# Autodesk Inventor assembly: proxxon_assembly
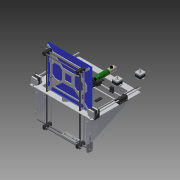
[picture p0: Inventor's stored thumbnail of the model, 180x180]
Saved by Autodesk Inventor 2013 (Build 170138000, 138)
## iProperties
Created: 2013-11-17
Part Number: proxxon_assembly
Document SubType Name: Assembly
Designer: Masta
Author: Masta
## Documents named in this file (24)
- D:\prusa i3\assembly\proxxon_assembly.iam
- D:\prusa i3\assembly\lasercut_aluminium\caddy.ipt
- D:\prusa i3\assembly\lasercut_aluminium\main_frame.ipt
- D:\prusa i3\assembly\lasercut_aluminium\side_frame.ipt
- D:\prusa i3\assembly\other\fi8x320.ipt
- D:\prusa i3\assembly\other\fi8x500.ipt
- D:\prusa i3\assembly\other\M5x300.ipt
- D:\prusa i3\assembly\other\M10x530.ipt
- D:\prusa i3\assembly\other\haetbed300.ipt
- D:\prusa i3\assembly\plastics\Y_corner.ipt
- D:\prusa i3\assembly\other\M8x290.ipt
- D:\prusa i3\assembly\other\M8x410.ipt
- D:\prusa i3\assembly\other\LM08UU.ipt
- D:\prusa i3\assembly\plastics\Prusa_i3_X_Carriage_Belt_Clamp.ipt
- D:\prusa i3\assembly\plastics\Prusa_i3_Y_Idler.ipt
- D:\prusa i3\assembly\other\nema17.ipt
- D:\prusa i3\assembly\old_parts_plastics\Prusa_i3_X_End_Idler.ipt
- D:\prusa i3\assembly\old_parts_plastics\Prusa_i3_X_End_Motor.ipt
- D:\prusa i3\assembly\old_parts_plastics\z-axis.ipt
- D:\prusa i3\assembly\old_parts_plastics\z-axis2.ipt
- D:\prusa i3\assembly\old_parts_plastics\x-carriage-24to30-gt2.ipt
- D:\prusa i3\assembly\plastics\adapter_50mm.ipt
- D:\prusa i3\assembly\old_parts_plastics\proxxon_mount.ipt
- D:\prusa i3\assembly\other\proxxon.ipt
## Components (48 placed, 23 different names)
1. main_frame:1 — Mate:1, Flush:3, Mate:2, Mate:3, Insert:1, Insert:2, Mate:12, Mate:13, Mate:14, Insert:10, Insert:11, Insert:12, Insert:13, Angle:6, Angle:7, Angle:8
2. caddy:1 — Insert:4, Insert:5, Tangent:26, Mate:9, Tangent:27, Tangent:30, Tangent:31, Mate:10, Tangent:32, Tangent:33, Mate:11, Mate:12, Mate:15
3. side_frame:1 — Flush:1, Flush:2, Flush:3, Mate:3, Flush:9
4. side_frame:2 — Flush:1, Mate:1, Flush:2, Mate:2, Zestawiający:22, Zestawiający:23
5. fi8x320:1 — Tangent:43, Insert:21
6. fi8x320:2 — Insert:19
7. fi8x500:1 — Tangent:18, Tangent:19, Mate:7, Mate:8
8. fi8x500:2 — Tangent:16, Tangent:17, Mate:5, Mate:6
9. fi8x500:3 — Tangent:38, Tangent:39, Tangent:40, Flush:13
10. fi8x500:4 — Tangent:41, Tangent:42, Flush:14, Insert:22
11. M10x530:1 — Insert:1, Tangent:10, Tangent:11, Tangent:12, Tangent:13, Flush:7
12. M10x530:2 — Insert:2, Tangent:8, Tangent:9, Tangent:14, Tangent:15
13. haetbed300:1 — Insert:4, Insert:5, Mate:13
14. Y_corner:1 — Tangent:6, Angle:2, Tangent:12, Tangent:13, Tangent:18, Tangent:19, Mate:7, Flush:6, Flush:7, Angle:5
15. Y_corner:2 — Tangent:5, Flush:5, Tangent:7, Angle:1, Tangent:14, Tangent:15, Tangent:16, Tangent:17, Mate:5, Flush:6, Tangent:20, Tangent:21
16. Y_corner:3 — Angle:4, Tangent:10, Tangent:11, Mate:8, Mate:15
17. Y_corner:4 — Angle:3, Tangent:8, Tangent:9, Mate:6, Tangent:22, Tangent:23, Tangent:24, Tangent:25
18. M8x290:1 — Tangent:5, Tangent:6, Flush:5, Tangent:7, Flush:8, Tangent:28, Tangent:29
19. M8x290:2 — Tangent:24, Tangent:25, Flush:10
20. M8x290:3 — Tangent:20, Tangent:21, Flush:8, Flush:10
21. M8x410:1 — Tangent:22, Tangent:23, Flush:9
22. LM08UU:1 — Tangent:44, Tangent:48, Mate:17
23. LM08UU:2 — Insert:9
24. LM08UU:3 — Tangent:26, Mate:9, Tangent:27
25. LM08UU:4 — Insert:8, Tangent:36, Tangent:37, Flush:12, Insert:20
26. LM08UU:5 — Tangent:46, Tangent:49, Mate:18
27. LM08UU:6 — Tangent:32, Tangent:33, Mate:11
28. LM08UU:7 — Insert:9, Tangent:34, Tangent:35, Flush:11, Tangent:43
29. LM08UU:8 — Tangent:45, Tangent:47, Mate:16, Insert:22
30. LM08UU:9 — Insert:8
31. LM08UU:10 — Tangent:30, Tangent:31, Mate:10
32. Prusa_i3_X_Carriage_Belt_Clamp:1
33. Prusa_i3_Y_Idler:1 — Tangent:28, Tangent:29, Angle:5
34. nema17:1 — Insert:6, Insert:17, Insert:18
35. nema17:2
36. nema17:3 — Insert:7, Insert:14, Insert:15
37. nema17:4
38. M5x300:3 — Insert:7
39. M5x300:4 — Insert:6
40. Prusa_i3_X_End_Idler:1 — Tangent:34, Tangent:35, Flush:11, Angle:7, Tangent:40, Flush:13, Tangent:41, Tangent:42, Flush:14
41. Prusa_i3_X_End_Motor:1 — Tangent:36, Tangent:37, Flush:12, Angle:6, Tangent:38, Tangent:39
42. z-axis:1 — Insert:10, Insert:11, Insert:17, Insert:18, Insert:19, Insert:20
43. z-axis2:1 — Insert:12, Insert:13, Insert:14, Insert:15, Insert:21
44. x-carriage-24to30-gt2:1 — Tangent:44, Tangent:45, Tangent:46, Tangent:47, Tangent:48, Tangent:49, Mate:16, Mate:17, Mate:18, Angle:8, Insert:23, Insert:24
45. adapter_50mm:1 — Zestawiający:22, Zestawiający:23
46. adapter_50mm:2
47. proxxon_mount:1 — Insert:23, Insert:24, Insert:25
48. proxxon:1 — Insert:25
## Relationships (108: Tangent 45, Insert 23, Mate 19, Flush 13, Angle 8)
- Flush:1: side_frame:1 ↔ side_frame:2
- Mate:1: main_frame:1 ↔ side_frame:2
- Flush:2: side_frame:1 ↔ side_frame:2
- Flush:3: main_frame:1 ↔ side_frame:1
- Mate:2 (0.25 mm): main_frame:1 ↔ side_frame:2
- Mate:3 (0.25 mm): main_frame:1 ↔ side_frame:1
- Insert:1 (-250 mm): main_frame:1 ↔ M10x530:1
- Insert:2 (-250 mm): main_frame:1 ↔ M10x530:2
- Insert:4 (10 mm): caddy:1 ↔ haetbed300:1
- Insert:5 (10 mm): caddy:1 ↔ haetbed300:1
- Tangent:5: Y_corner:2 ↔ M8x290:1
- Tangent:6: Y_corner:1 ↔ M8x290:1
- Flush:5 (-11 mm): Y_corner:2 ↔ M8x290:1
- Tangent:7: Y_corner:2 ↔ M8x290:1
- Angle:1 (0 deg): Y_corner:2
- Angle:2 (0 deg): Y_corner:1
- Angle:3 (180 deg): Y_corner:4
- Angle:4 (0 deg): Y_corner:3
- Tangent:8: M10x530:2 ↔ Y_corner:4
- Tangent:9: M10x530:2 ↔ Y_corner:4
- Tangent:10: M10x530:1 ↔ Y_corner:3
- Tangent:11: M10x530:1 ↔ Y_corner:3
- Tangent:12: M10x530:1 ↔ Y_corner:1
- Tangent:13: M10x530:1 ↔ Y_corner:1
- Tangent:14: M10x530:2 ↔ Y_corner:2
- Tangent:15: M10x530:2 ↔ Y_corner:2
- Tangent:16: fi8x500:2 ↔ Y_corner:2
- Tangent:17: fi8x500:2 ↔ Y_corner:2
- Mate:5: fi8x500:2 ↔ Y_corner:2
- Mate:6: fi8x500:2 ↔ Y_corner:4
- Tangent:18: fi8x500:1 ↔ Y_corner:1
- Tangent:19: fi8x500:1 ↔ Y_corner:1
- Mate:7: fi8x500:1 ↔ Y_corner:1
- Mate:8: fi8x500:1 ↔ Y_corner:3
- Flush:6: Y_corner:1 ↔ Y_corner:2
- Flush:7 (13 mm): M10x530:1 ↔ Y_corner:1
- Tangent:20: Y_corner:2 ↔ M8x290:3
- Tangent:21: Y_corner:2 ↔ M8x290:3
- Flush:8: M8x290:1 ↔ M8x290:3
- Tangent:22: Y_corner:4 ↔ M8x410:1
- Tangent:23: Y_corner:4 ↔ M8x410:1
- Flush:9 (-11 mm): side_frame:1 ↔ M8x410:1
- Tangent:24: Y_corner:4 ↔ M8x290:2
- Tangent:25: Y_corner:4 ↔ M8x290:2
- Flush:10: M8x290:2 ↔ M8x290:3
- Tangent:26: caddy:1 ↔ LM08UU:3
- Mate:9: caddy:1 ↔ LM08UU:3
- Tangent:27: caddy:1 ↔ LM08UU:3
- Tangent:28: M8x290:1 ↔ Prusa_i3_Y_Idler:1
- Tangent:29: M8x290:1 ↔ Prusa_i3_Y_Idler:1
- Angle:5 (0 deg): Y_corner:1 ↔ Prusa_i3_Y_Idler:1
- Tangent:30: caddy:1 ↔ LM08UU:10
- Tangent:31: caddy:1 ↔ LM08UU:10
- Mate:10: caddy:1 ↔ LM08UU:10
- Tangent:32: caddy:1 ↔ LM08UU:6
- Tangent:33: caddy:1 ↔ LM08UU:6
- Mate:11: caddy:1 ↔ LM08UU:6
- Mate:12 (16.5 mm): main_frame:1 ↔ caddy:1
- Mate:13 (15 mm): main_frame:1 ↔ haetbed300:1
- Mate:14: main_frame:1
- Mate:15 (340 mm): caddy:1 ↔ Y_corner:3
- Insert:6: nema17:1 ↔ M5x300:4
- Insert:7: nema17:3 ↔ M5x300:3
- Insert:8 (12 mm): LM08UU:4 ↔ LM08UU:9
- Insert:9 (12 mm): LM08UU:2 ↔ LM08UU:7
- Tangent:34: LM08UU:7 ↔ Prusa_i3_X_End_Idler:1
- Tangent:35: LM08UU:7 ↔ Prusa_i3_X_End_Idler:1
- Flush:11: LM08UU:7 ↔ Prusa_i3_X_End_Idler:1
- Tangent:36: LM08UU:4 ↔ Prusa_i3_X_End_Motor:1
- Tangent:37: LM08UU:4 ↔ Prusa_i3_X_End_Motor:1
- Flush:12: LM08UU:4 ↔ Prusa_i3_X_End_Motor:1
- Insert:10: main_frame:1 ↔ z-axis:1
- Insert:11: main_frame:1 ↔ z-axis:1
- Insert:12: main_frame:1 ↔ z-axis2:1
- Insert:13: main_frame:1 ↔ z-axis2:1
- Insert:14 (4.5 mm): nema17:3 ↔ z-axis2:1
- Insert:15 (4.5 mm): nema17:3 ↔ z-axis2:1
- Insert:17 (4.5 mm): nema17:1 ↔ z-axis:1
- Insert:18 (4.5 mm): nema17:1 ↔ z-axis:1
- Insert:19 (-4.5 mm): fi8x320:2 ↔ z-axis:1
- Insert:20: LM08UU:4 ↔ z-axis:1
- Angle:6 (180 deg): main_frame:1 ↔ Prusa_i3_X_End_Motor:1
- Angle:7 (180 deg): main_frame:1 ↔ Prusa_i3_X_End_Idler:1
- Tangent:38: fi8x500:3 ↔ Prusa_i3_X_End_Motor:1
- Tangent:39: fi8x500:3 ↔ Prusa_i3_X_End_Motor:1
- Tangent:40: fi8x500:3 ↔ Prusa_i3_X_End_Idler:1
- Flush:13: fi8x500:3 ↔ Prusa_i3_X_End_Idler:1
- Tangent:41: fi8x500:4 ↔ Prusa_i3_X_End_Idler:1
- Tangent:42: fi8x500:4 ↔ Prusa_i3_X_End_Idler:1
- Flush:14: fi8x500:4 ↔ Prusa_i3_X_End_Idler:1
- Tangent:43: fi8x320:1 ↔ LM08UU:7
- Insert:21 (-4.5 mm): fi8x320:1 ↔ z-axis2:1
- Tangent:44: LM08UU:1 ↔ x-carriage-24to30-gt2:1
- Tangent:45: LM08UU:8 ↔ x-carriage-24to30-gt2:1
- Tangent:46: LM08UU:5 ↔ x-carriage-24to30-gt2:1
- Tangent:47: LM08UU:8 ↔ x-carriage-24to30-gt2:1
- Tangent:48: LM08UU:1 ↔ x-carriage-24to30-gt2:1
- Tangent:49: LM08UU:5 ↔ x-carriage-24to30-gt2:1
- Mate:16: LM08UU:8 ↔ x-carriage-24to30-gt2:1
- Mate:17: LM08UU:1 ↔ x-carriage-24to30-gt2:1
- Mate:18: LM08UU:5 ↔ x-carriage-24to30-gt2:1
- Insert:22 (380 mm): fi8x500:4 ↔ LM08UU:8
- Angle:8 (0 deg): main_frame:1 ↔ x-carriage-24to30-gt2:1
- Zestawiający:22 [Mate]: side_frame:2 ↔ adapter_50mm:1
- Zestawiający:23 [Mate]: side_frame:2 ↔ adapter_50mm:1
- Insert:23: x-carriage-24to30-gt2:1 ↔ proxxon_mount:1
- Insert:24: x-carriage-24to30-gt2:1 ↔ proxxon_mount:1
- Insert:25: proxxon_mount:1 ↔ proxxon:1
